# Autodesk Inventor assembly: 剪刀式升降
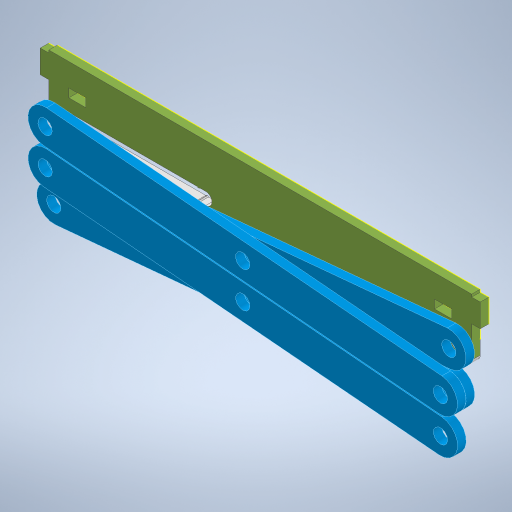
[picture p0: Inventor's stored thumbnail of the model, 512x512]
Saved by Autodesk Inventor 2023 (Build 270158000, 158)
## iProperties
Created: 2023-03-17
Part Number: 剪刀式升降
Document SubType Name: Assembly
Designer: may9c
Author: may9c
## Documents named in this file (3)
- E:\1112\實務\升降\剪刀式升降.iam
- E:\1112\實務\升降\連桿.ipt
- E:\1112\實務\升降\chassis_1_2_1.ipt
## Components (5 placed, 2 different names)
1. 連桿:1 — 插入:1, 插入:2, 插入:4
2. chassis_1_2_1:1 — 貼合:1, 貼合:2, 插入:1, 相切:1
3. 連桿:2 — 插入:2, 插入:3, 相切:1
4. 連桿:3 — 插入:3, 插入:5
5. 連桿:4 — 插入:4, 插入:5
## Relationships (8: Insert 5, Mate 2, Tangent 1)
- 貼合:1 [Mate]: chassis_1_2_1:1
- 貼合:2 [Mate]: chassis_1_2_1:1
- 插入:1 [Insert]: 連桿:1 ↔ chassis_1_2_1:1
- 插入:2 [Insert]: 連桿:1 ↔ 連桿:2
- 插入:3 [Insert]: 連桿:2 ↔ 連桿:3
- 插入:4 [Insert]: 連桿:1 ↔ 連桿:4
- 插入:5 [Insert]: 連桿:3 ↔ 連桿:4
- 相切:1 [Tangent]: chassis_1_2_1:1 ↔ 連桿:2
